# Autodesk Inventor assembly: base
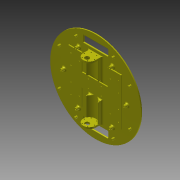
[picture p0: Inventor's stored thumbnail of the model, 180x180]
Saved by Autodesk Inventor 2015 (Build 190159000, 159)
## iProperties
Created: 2015-03-17
Part Number: base
Document SubType Name: Assembly
Designer: david_000
Author: david_000
## Documents named in this file (4)
- C:\Users\david_000\Dropbox\minibot\mechanics\base.iam
- C:\Users\david_000\Dropbox\minibot\mechanics\base_1.ipt
- C:\Users\david_000\Dropbox\minibot\mechanics\base_2.ipt
- C:\Users\david_000\Dropbox\minibot\mechanics\base_3.ipt
## Components (5 placed, 3 different names)
1. base_3:1 — Coincidencia:7, Coincidencia:8, Coincidencia:9, Coincidencia:10, Coincidencia:11, Coincidencia:12, Coincidencia:13, Coincidencia:14, Coincidencia:15
2. base_1:3 — Coincidencia:7, Coincidencia:8, Coincidencia:9, Nivelación:1, Nivelación:2
3. base_1:4 — Coincidencia:10, Coincidencia:11, Nivelación:1
4. base_2:3 — Nivelación:3, Coincidencia:14, Coincidencia:15
5. base_2:4 — Coincidencia:12, Coincidencia:13, Nivelación:2, Nivelación:3
## Relationships (12: Mate 9, Flush 3)
- Coincidencia:7 [Mate]: base_3:1 ↔ base_1:3
- Coincidencia:8 [Mate]: base_3:1 ↔ base_1:3
- Coincidencia:9 [Mate]: base_3:1 ↔ base_1:3
- Coincidencia:10 [Mate]: base_3:1 ↔ base_1:4
- Coincidencia:11 [Mate]: base_3:1 ↔ base_1:4
- Nivelación:1 [Flush]: base_1:3 ↔ base_1:4
- Coincidencia:12 [Mate]: base_3:1 ↔ base_2:4
- Coincidencia:13 [Mate]: base_3:1 ↔ base_2:4
- Nivelación:2 [Flush]: base_1:3 ↔ base_2:4
- Nivelación:3 [Flush]: base_2:3 ↔ base_2:4
- Coincidencia:14 [Mate]: base_3:1 ↔ base_2:3
- Coincidencia:15 [Mate]: base_3:1 ↔ base_2:3
